# Autodesk Inventor assembly: Bar Back Cabinet
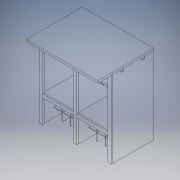
[picture p0: Inventor's stored thumbnail of the model, 180x180]
Saved by Autodesk Inventor 2016 (Build 200138000, 138)
## iProperties
Created: 2017-11-04
Part Number: Bar Back Cabinet
Document SubType Name: Assembly
Designer: mathaetaes
Author: mathaetaes
## Documents named in this file (16)
- E:\Projects\3D Printer\printer projects\My Designs\Bar Cabinet 2.2.2018\Bar Back Cabinet.iam
- E:\Projects\3D Printer\printer projects\My Designs\Bar Cabinet 2.2.2018\Left Side.ipt
- E:\Projects\3D Printer\printer projects\My Designs\Bar Cabinet 2.2.2018\Right Side.ipt
- E:\Projects\3D Printer\printer projects\My Designs\Bar Cabinet 2.2.2018\Vertical Shelf.ipt
- E:\Projects\3D Printer\printer projects\My Designs\Bar Cabinet 2.2.2018\Top.ipt
- E:\Projects\3D Printer\printer projects\My Designs\Bar Cabinet 2.2.2018\Wine Bottle Rack Back Panel.ipt
- E:\Projects\3D Printer\printer projects\My Designs\Bar Cabinet 2.2.2018\Back Panel Bottom.ipt
- E:\Projects\3D Printer\printer projects\My Designs\Bar Cabinet 2.2.2018\Wine Rack Assembly.iam
- E:\Projects\3D Printer\printer projects\My Designs\Bar Cabinet 2.2.2018\Horizontal Shelf.ipt
- E:\Projects\3D Printer\printer projects\My Designs\Bar Cabinet 2.2.2018\Wine Rack and Light Shelf Assembly Left.iam
- E:\Projects\3D Printer\printer projects\My Designs\Bar Cabinet 2.2.2018\Wine Rack and Light Shelf Assembly Right.iam
- E:\Projects\3D Printer\printer projects\My Designs\Bar Cabinet 2.2.2018\Cabinet Support Frame Side Vertical Bar.ipt
- E:\Projects\3D Printer\printer projects\My Designs\Bar Cabinet 2.2.2018\Cabinet Support Frame Center Vertical Bar.ipt
- E:\Projects\3D Printer\printer projects\My Designs\Bar Cabinet 2.2.2018\Cabinet Support Frame Horizontal Bar Notcked.ipt
- E:\Projects\3D Printer\printer projects\My Designs\Bar Cabinet 2.2.2018\Glue-on .25in post to make up for our mistake.ipt
- E:\Projects\3D Printer\printer projects\My Designs\Bar Cabinet 2.2.2018\Cabinet Back Sheet.ipt
## Components (21 placed, 15 different names)
1. Back Panel Bottom:1 — Mate:37, Mate:38, Mate:76
2. Back Panel Bottom:2 — Mate:33, Mate:35, Mate:77
3. Top:1 — Mate:1, Mate:2, Mate:3, Mate:4, Mate:5, Mate:6, Mate:7, Mate:9, Mate:53, Mate:54, Mate:61, Mate:78
4. Left Side:1 — Mate:1, Mate:2, Mate:3, Mate:13, Mate:15, Mate:19, Mate:29, Mate:30, Flush:3, Mate:37, Mate:52, Flush:6, Mate:57, Mate:58, Mate:59, Mate:63, Mate:73, Mate:77
5. Right Side:1 — Mate:4, Mate:5, Mate:6, Mate:24, Mate:25, Mate:31, Mate:32, Mate:33, Mate:51, Flush:5, Mate:55, Mate:64, Mate:76, Mate:82
6. Vertical Shelf:1 — Mate:7, Mate:9, Mate:16, Mate:17, Flush:1, Mate:22, Flush:2, Flush:4, Mate:56, Mate:62, Mate:72, Mate:74, Mate:78, Mate:79, Mate:80, Flush:9, Mate:81
7. Wine Rack Assembly:1 [sub-assembly] — Mate:13, Mate:15, Mate:57, Mate:58, Mate:59
8. Wine Rack Assembly:2 [sub-assembly] — Mate:16, Mate:17, Mate:55
9. Horizontal Shelf:1 — Mate:19, Flush:1, Mate:38, Mate:63, Mate:71, Flush:8
10. Horizontal Shelf:2 — Mate:22, Flush:2, Mate:23, Mate:35, Mate:64, Mate:65, Mate:67, Flush:7, Mate:75
11. Wine Bottle Rack Back Panel:3 — Mate:23, Mate:24, Mate:25
12. Wine Bottle Rack Back Panel:4 — Mate:71, Mate:72, Mate:73
13. Wine Rack and Light Shelf Assembly Right:1 [sub-assembly] — Mate:31, Mate:32, Flush:4
14. Wine Rack and Light Shelf Assembly Left:1 [sub-assembly] — Mate:29, Mate:30, Flush:3, Mate:56, Mate:79, Mate:80, Flush:9
15. Cabinet Support Frame Side Bar:1 — Mate:51, Mate:54, Flush:5
16. Cabinet Support Frame Side Bar:2 — Mate:52, Mate:53, Flush:6, Mate:60, Mate:66
17. Cabinet Support Frame Horizontal Bar Notcked:1 — Mate:60, Mate:61, Mate:62, Mate:68, Mate:69
18. Cabinet Support Frame Horizontal Bar Notcked:2 — Mate:65, Mate:66, Mate:67, Flush:7, Mate:70
19. Cabinet Support Frame Center Vertical Bar:1 — Mate:68, Mate:69, Mate:70
20. Glue-on .25in post to make up for our mistake:1 — Mate:74, Flush:8, Mate:75, Mate:83
21. Cabinet Back Sheet:1 — Mate:81, Mate:82, Mate:83
## Relationships (67: Mate 58, Flush 9)
- Mate:1: Top:1 ↔ Left Side:1
- Mate:2: Top:1 ↔ Left Side:1
- Mate:3: Top:1 ↔ Left Side:1
- Mate:4: Top:1 ↔ Right Side:1
- Mate:5: Top:1 ↔ Right Side:1
- Mate:6: Top:1 ↔ Right Side:1
- Mate:7: Top:1 ↔ Vertical Shelf:1
- Mate:9: Top:1 ↔ Vertical Shelf:1
- Mate:13: Left Side:1 ↔ Wine Rack Assembly:1
- Mate:15: Left Side:1 ↔ Wine Rack Assembly:1
- Mate:16: Vertical Shelf:1 ↔ Wine Rack Assembly:2
- Mate:17: Vertical Shelf:1 ↔ Wine Rack Assembly:2
- Mate:19: Left Side:1 ↔ Horizontal Shelf:1
- Flush:1: Vertical Shelf:1 ↔ Horizontal Shelf:1
- Mate:22: Vertical Shelf:1 ↔ Horizontal Shelf:2
- Flush:2: Vertical Shelf:1 ↔ Horizontal Shelf:2
- Mate:23: Horizontal Shelf:2 ↔ Wine Bottle Rack Back Panel:3
- Mate:24: Right Side:1 ↔ Wine Bottle Rack Back Panel:3
- Mate:25: Right Side:1 ↔ Wine Bottle Rack Back Panel:3
- Mate:29: Left Side:1 ↔ Wine Rack and Light Shelf Assembly Left:1
- Mate:30: Left Side:1 ↔ Wine Rack and Light Shelf Assembly Left:1
- Flush:3: Left Side:1 ↔ Wine Rack and Light Shelf Assembly Left:1
- Mate:31: Right Side:1 ↔ Wine Rack and Light Shelf Assembly Right:1
- Mate:32: Right Side:1 ↔ Wine Rack and Light Shelf Assembly Right:1
- Flush:4: Vertical Shelf:1 ↔ Wine Rack and Light Shelf Assembly Right:1
- Mate:33: Back Panel Bottom:2 ↔ Right Side:1
- Mate:35: Back Panel Bottom:2 ↔ Horizontal Shelf:2
- Mate:37: Back Panel Bottom:1 ↔ Left Side:1
- Mate:38: Back Panel Bottom:1 ↔ Horizontal Shelf:1
- Mate:51: Right Side:1 ↔ Cabinet Support Frame Side Bar:1
- Mate:52: Left Side:1 ↔ Cabinet Support Frame Side Bar:2
- Mate:53: Top:1 ↔ Cabinet Support Frame Side Bar:2
- Mate:54: Top:1 ↔ Cabinet Support Frame Side Bar:1
- Flush:5: Right Side:1 ↔ Cabinet Support Frame Side Bar:1
- Flush:6: Left Side:1 ↔ Cabinet Support Frame Side Bar:2
- Mate:55: Right Side:1 ↔ Wine Rack Assembly:2
- Mate:56: Vertical Shelf:1 ↔ Wine Rack and Light Shelf Assembly Left:1
- Mate:57: Left Side:1 ↔ Wine Rack Assembly:1
- Mate:58: Left Side:1 ↔ Wine Rack Assembly:1
- Mate:59: Left Side:1 ↔ Wine Rack Assembly:1
- Mate:60: Cabinet Support Frame Side Bar:2 ↔ Cabinet Support Frame Horizontal Bar Notcked:1
- Mate:61: Top:1 ↔ Cabinet Support Frame Horizontal Bar Notcked:1
- Mate:62: Vertical Shelf:1 ↔ Cabinet Support Frame Horizontal Bar Notcked:1
- Mate:63: Left Side:1 ↔ Horizontal Shelf:1
- Mate:64: Right Side:1 ↔ Horizontal Shelf:2
- Mate:65: Horizontal Shelf:2 ↔ Cabinet Support Frame Horizontal Bar Notcked:2
- Mate:66: Cabinet Support Frame Side Bar:2 ↔ Cabinet Support Frame Horizontal Bar Notcked:2
- Mate:67: Horizontal Shelf:2 ↔ Cabinet Support Frame Horizontal Bar Notcked:2
- Flush:7 (-6.35 mm): Horizontal Shelf:2 ↔ Cabinet Support Frame Horizontal Bar Notcked:2
- Mate:68: Cabinet Support Frame Horizontal Bar Notcked:1 ↔ Cabinet Support Frame Center Vertical Bar:1
- Mate:69: Cabinet Support Frame Horizontal Bar Notcked:1 ↔ Cabinet Support Frame Center Vertical Bar:1
- Mate:70: Cabinet Support Frame Horizontal Bar Notcked:2 ↔ Cabinet Support Frame Center Vertical Bar:1
- Mate:71: Horizontal Shelf:1 ↔ Wine Bottle Rack Back Panel:4
- Mate:72: Vertical Shelf:1 ↔ Wine Bottle Rack Back Panel:4
- Mate:73: Left Side:1 ↔ Wine Bottle Rack Back Panel:4
- Mate:74: Vertical Shelf:1 ↔ Glue-on .25in post to make up for our mistake:1
- Flush:8: Horizontal Shelf:1 ↔ Glue-on .25in post to make up for our mistake:1
- Mate:75: Horizontal Shelf:2 ↔ Glue-on .25in post to make up for our mistake:1
- Mate:76: Back Panel Bottom:1 ↔ Right Side:1
- Mate:77: Back Panel Bottom:2 ↔ Left Side:1
- Mate:78: Top:1 ↔ Vertical Shelf:1
- Mate:79: Vertical Shelf:1 ↔ Wine Rack and Light Shelf Assembly Left:1
- Mate:80: Vertical Shelf:1 ↔ Wine Rack and Light Shelf Assembly Left:1
- Flush:9: Vertical Shelf:1 ↔ Wine Rack and Light Shelf Assembly Left:1
- Mate:81: Vertical Shelf:1 ↔ Cabinet Back Sheet:1
- Mate:82: Right Side:1 ↔ Cabinet Back Sheet:1
- Mate:83: Glue-on .25in post to make up for our mistake:1 ↔ Cabinet Back Sheet:1
